# Autodesk Inventor assembly: intake_gearbox
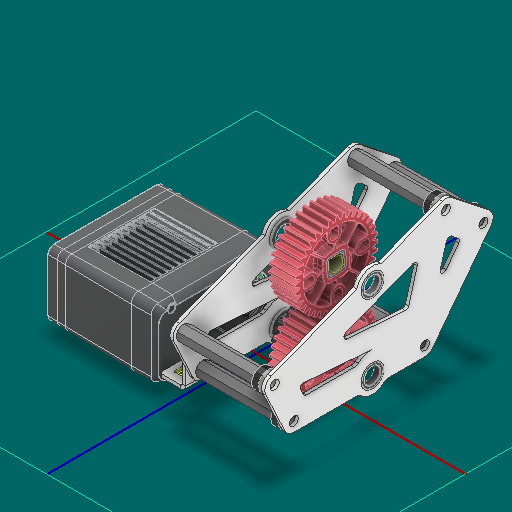
[picture p0: Inventor's stored thumbnail of the model, 512x512]
Saved by Autodesk Inventor 2025 (Build 290162000, 162)
## iProperties
Created: 2024-07-02
Part Number: intake_gearbox
Document SubType Name: Assembly
Designer: Averey Ku
Author: Averey Ku
## Documents named in this file (15)
- C:\Users\avere\vex_robotics_high_stakes\hardware\cad\EARLY_SEASON\tower\intake_gearbox.iam
- C:\Users\avere\vex_robotics_high_stakes\hardware\cad\VEX-CAD-Inventor\Motion\Gears\HS Gear\HS 36T Gear, No Insert.iam
- C:\Users\avere\vex_robotics_high_stakes\hardware\cad\VEX-CAD-Inventor\Structure\Angle\Aluminum 1x1\Alu Angle 1x1x6.ipt
- C:\Users\avere\vex_robotics_high_stakes\hardware\cad\EARLY_SEASON\tower\custom_parts\gearbox_gusset.ipt
- C:\Users\avere\vex_robotics_high_stakes\hardware\cad\VEX-CAD-Inventor\Motion\Shaft HS\HS Bushing 0.1250.ipt
- C:\Users\avere\vex_robotics_high_stakes\hardware\cad\VEX-CAD-Inventor\Electronics\V5 Motor.ipt
- C:\Users\avere\vex_robotics_high_stakes\hardware\cad\VEX-CAD-Inventor\Motion\Sprockets\6P Sprocket\6P 8T Sprocket, No Insert.iam
- C:\Users\avere\vex_robotics_high_stakes\hardware\cad\VEX-CAD-Inventor\Structure\Standoff\Standoff 1.50.ipt
- C:\Users\avere\vex_robotics_high_stakes\hardware\cad\VEX-CAD-Inventor\Motion\Spacers\Spacer Nylon .375 OD\NSpacer .375 OD x .125.ipt
- C:\Users\avere\vex_robotics_high_stakes\hardware\cad\VEX-CAD-Inventor\Motion\Spacers\Washer Steel\SWasher .375 OD x .062500.ipt
- C:\Users\avere\vex_robotics_high_stakes\hardware\cad\VEX-CAD-Inventor\Motion\Gears\HS Gear.iam
- C:\Users\avere\vex_robotics_high_stakes\hardware\cad\VEX-CAD-Inventor\Motion\Sprockets\6P Sprocket.iam
- C:\Users\avere\vex_robotics_high_stakes\hardware\cad\VEX-CAD-Inventor\Structure\Standoff.ipt
- C:\Users\avere\vex_robotics_high_stakes\hardware\cad\VEX-CAD-Inventor\Motion\Spacers\Spacer Nylon .375 OD.ipt
- C:\Users\avere\vex_robotics_high_stakes\hardware\cad\VEX-CAD-Inventor\Motion\Spacers\Washer Steel.ipt
## Components (26 placed, 9 different names)
1. HS 36T Gear, No Insert:1 [sub-assembly]
2. HS 36T Gear, No Insert:2 [sub-assembly]
3. Alu Angle 1x1x6:1
4. gearbox_gusset:1
5. gearbox_gusset:2 — Insert:11, Insert:12, Insert:13, Insert:14, Insert:15
6. HS Bushing 0.1250:1
7. HS Bushing 0.1250:2
8. HS Bushing 0.1250:3
9. HS Bushing 0.1250:4
10. V5 Motor:1
11. 6P 8T Sprocket, No Insert:1 [sub-assembly]
12. Standoff 1.50:1 — Insert:11, Insert:22
13. Standoff 1.50:2 — Insert:12, Insert:23
14. Standoff 1.50:3 — Insert:13, Insert:20
15. Standoff 1.50:4 — Insert:14, Insert:21
16. Standoff 1.50:5 — Insert:15, Insert:25
17. NSpacer .375 OD x .125:1 — Insert:17, Insert:22
18. NSpacer .375 OD x .125:2 — Insert:19, Insert:20
19. NSpacer .375 OD x .125:3 — Insert:16, Insert:21
20. NSpacer .375 OD x .125:4 — Insert:18, Insert:23
21. SWasher .375 OD x .062500:1 — Insert:18
22. SWasher .375 OD x .062500:2 — Insert:16
23. SWasher .375 OD x .062500:3 — Insert:19
24. SWasher .375 OD x .062500:4 — Insert:17
25. NSpacer .375 OD x .125:5 — Insert:25
26. SWasher .375 OD x .062500:5
## Relationships (28: Insert 25, Mate 3)
- [Mate]: gearbox_gusset:1 ↔ gearbox_gusset:2
- [Insert]: gearbox_gusset:2 ↔ HS Bushing 0.1250:1
- [Insert]: gearbox_gusset:1 ↔ HS Bushing 0.1250:2
- [Insert]: gearbox_gusset:1 ↔ HS Bushing 0.1250:3
- [Insert]: gearbox_gusset:2 ↔ HS Bushing 0.1250:4
- [Insert] (42.8625 mm): gearbox_gusset:1 ↔ gearbox_gusset:2
- [Insert]: Alu Angle 1x1x6:1 ↔ gearbox_gusset:2
- [Mate]: Alu Angle 1x1x6:1 ↔ gearbox_gusset:2
- [Insert] (12.7 mm): HS 36T Gear, No Insert:2 ↔ HS Bushing 0.1250:1
- [Insert]: Alu Angle 1x1x6:1 ↔ V5 Motor:1
- [Mate]: Alu Angle 1x1x6:1 ↔ V5 Motor:1
- [Insert] (12.7 mm): HS 36T Gear, No Insert:1 ↔ HS Bushing 0.1250:4
- [Insert]: HS 36T Gear, No Insert:2 ↔ 6P 8T Sprocket, No Insert:1
- Insert:11: gearbox_gusset:2 ↔ Standoff 1.50:1
- Insert:12: gearbox_gusset:2 ↔ Standoff 1.50:2
- Insert:13: gearbox_gusset:2 ↔ Standoff 1.50:3
- Insert:14: gearbox_gusset:2 ↔ Standoff 1.50:4
- Insert:15: gearbox_gusset:2 ↔ Standoff 1.50:5
- Insert:16: NSpacer .375 OD x .125:3 ↔ SWasher .375 OD x .062500:2
- Insert:17: NSpacer .375 OD x .125:1 ↔ SWasher .375 OD x .062500:4
- Insert:18: NSpacer .375 OD x .125:4 ↔ SWasher .375 OD x .062500:1
- Insert:19: NSpacer .375 OD x .125:2 ↔ SWasher .375 OD x .062500:3
- Insert:20: Standoff 1.50:3 ↔ NSpacer .375 OD x .125:2
- Insert:21: Standoff 1.50:4 ↔ NSpacer .375 OD x .125:3
- Insert:22: Standoff 1.50:1 ↔ NSpacer .375 OD x .125:1
- Insert:23: Standoff 1.50:2 ↔ NSpacer .375 OD x .125:4
- [Insert]: NSpacer .375 OD x .125:5 ↔ SWasher .375 OD x .062500:5
- Insert:25: Standoff 1.50:5 ↔ NSpacer .375 OD x .125:5
## Named parameters: d40_d46 = 0 mm, d41_d48 = 0 mm, d26_d20 = 0 mm
